# Autodesk Inventor assembly: Colmeia
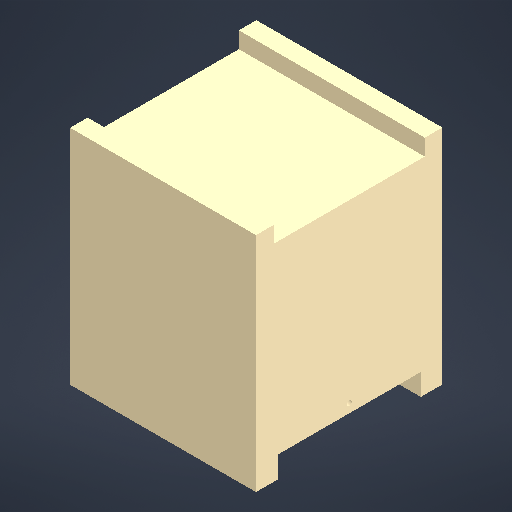
[picture p0: Inventor's stored thumbnail of the model, 512x512]
Saved by Autodesk Inventor 2027 (Build 310192060, 192F)
## iProperties
Created: 2026-10-01
Part Number: Colmeia
Document SubType Name: Assembly
Designer: EspacoMaker
Author: EspacoMaker
## Documents named in this file (5)
- C:\Users\notra\Desktop\BeeBox\3dFiles\Colmeia.iam
- C:\Users\notra\Desktop\BeeBox\3dFiles\FundoColmeia.ipt
- C:\Users\notra\Desktop\BeeBox\3dFiles\NinhoColmeia.ipt
- C:\Users\notra\Desktop\BeeBox\3dFiles\Melgueira-Sobreninho.ipt
- C:\Users\notra\Desktop\BeeBox\3dFiles\Tampa.ipt
## Components (5 placed, 4 different names)
1. FundoColmeia:1 — Mate:1, Flush:1, Flush:2
2. NinhoColmeia:1 — Mate:1, Flush:1, Flush:2, Mate:2, Flush:3, Flush:4
3. Melgueira-Sobreninho:1 — Mate:2, Flush:3, Flush:4, Mate:3, Flush:5, Flush:6
4. Melgueira-Sobreninho:2 — Mate:3, Flush:5, Flush:6, Mate:4, Flush:7, Flush:8
5. Tampa:1 — Mate:4, Flush:7, Flush:8
## Relationships (12: Flush 8, Mate 4)
- Mate:1: FundoColmeia:1 ↔ NinhoColmeia:1
- Flush:1: FundoColmeia:1 ↔ NinhoColmeia:1
- Flush:2: FundoColmeia:1 ↔ NinhoColmeia:1
- Mate:2: NinhoColmeia:1 ↔ Melgueira-Sobreninho:1
- Flush:3: NinhoColmeia:1 ↔ Melgueira-Sobreninho:1
- Flush:4: NinhoColmeia:1 ↔ Melgueira-Sobreninho:1
- Mate:3: Melgueira-Sobreninho:1 ↔ Melgueira-Sobreninho:2
- Flush:5: Melgueira-Sobreninho:1 ↔ Melgueira-Sobreninho:2
- Flush:6: Melgueira-Sobreninho:1 ↔ Melgueira-Sobreninho:2
- Mate:4: Melgueira-Sobreninho:2 ↔ Tampa:1
- Flush:7: Melgueira-Sobreninho:2 ↔ Tampa:1
- Flush:8: Melgueira-Sobreninho:2 ↔ Tampa:1
## Named parameters: Finish1_Area = 9696.18
note: some values were not read from the file. Shown as the stored number, unit unknown: "Finish1_Area".
